# Autodesk Inventor assembly: TestAssm
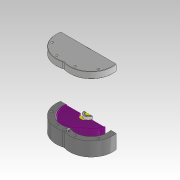
[picture p0: Inventor's stored thumbnail of the model, 180x180]
Saved by Autodesk Inventor 2020 (Build 240168000, 168)
## iProperties
Created: 2021-05-17
Part Number: TestAssm
Document SubType Name: Assembly
Designer: DDeGo
Author: DDeGo
## Documents named in this file (14)
- C:\Users\DDeGo\Documents\Drew\Projects\AirWankelEngine\cad\LiquidPiston V1\TestAssm.iam
- C:\Users\DDeGo\Documents\Drew\Projects\AirWankelEngine\cad\LiquidPiston V1\TestHousing.ipt
- C:\Users\DDeGo\Documents\Drew\Projects\AirWankelEngine\cad\LiquidPiston V1\TestRotor.ipt
- C:\Users\DDeGo\Documents\Drew\Projects\AirWankelEngine\cad\LiquidPiston V1\TestCam.ipt
- C:\Users\DDeGo\Documents\Drew\Projects\AirWankelEngine\cad\LiquidPiston V1\TestAssm\Design Accelerator\Spur Gears1.iam
- C:\Users\DDeGo\Documents\Drew\Projects\AirWankelEngine\cad\hardware\6701 bearing.ipt
- C:\Users\DDeGo\Documents\Drew\Projects\AirWankelEngine\cad\LiquidPiston V1\TestHead.ipt
- C:\Users\DDeGo\Documents\Drew\Projects\AirWankelEngine\cad\LiquidPiston V1\ApexSeal.ipt
- C:\Users\DDeGo\Documents\Drew\Projects\AirWankelEngine\cad\hardware\MR85 bearing.ipt
- C:\Users\DDeGo\Documents\Drew\Projects\AirWankelEngine\cad\LiquidPiston V1\TestRotorTeeth.ipt
- C:\Users\DDeGo\Documents\Drew\Projects\AirWankelEngine\cad\LiquidPiston V1\Flywheel.ipt
- C:\Users\DDeGo\Documents\Drew\Projects\AirWankelEngine\cad\hardware\oring_4x2x1.ipt
- C:\Users\DDeGo\Documents\Drew\Projects\AirWankelEngine\cad\hardware\2x22 pin.ipt
- C:\Users\DDeGo\Documents\Drew\Projects\AirWankelEngine\cad\LiquidPiston V1\ValveThing2.ipt
## Components (18 placed, 13 different names)
1. TestHousing:1 — Mate:2, Mate:11, Mate:14, Mate:15, Mate:20, Mate:21, Mate:65, Mate:66, Mate:67, Mate:68, Mate:69
2. TestRotor:1 — Mate:2, Mate:3, Rotation:1, Mate:5, Mate:29, Mate:30, Angle:1, Mate:42
3. TestCam:1 — Mate:3, Rotation:1, Mate:43, Mate:44, Mate:46, Mate:47, Mate:48, Flush:6
4. Spur Gears:1 [sub-assembly]
5. 6701 bearing:1 — Mate:5, Mate:42, Flush:6
6. ApexSeal:1 — Mate:11, Mate:67
7. ApexSeal:2 — Mate:14, Mate:68
8. ApexSeal:3 — Mate:15, Mate:66
9. MR85 bearing:1 — Mate:20, Mate:21, Mate:32, Mate:33
10. MR85 bearing:2 — Mate:46, Mate:48, Mate:64
11. TestRotorTeeth:1 — Mate:29, Mate:30, Angle:1
12. Flywheel:1 — Mate:32, Mate:33, Mate:45, Mate:47
13. oring_4x2x1:1 — Flush:2, Flush:3, Mate:71, Tangent:1
14. oring_4x2x1:2 — Flush:2, Mate:70, Tangent:2
15. oring_4x2x1:3 — Flush:3, Mate:72
16. 2x22 pin:1 — Mate:43, Mate:44, Mate:45
17. TestHead:1 — Mate:64, Mate:65, Mate:69, Mate:70, Mate:71, Mate:72, Tangent:1, Mate:73, Mate:74
18. ValveThing2:1 — Mate:73, Mate:74, Tangent:2
## Relationships (37: Mate 30, Flush 3, Tangent 2, RelateRotation 1, Angle 1)
- Mate:2 (-0.25 mm): TestHousing:1 ↔ TestRotor:1
- Mate:3: TestRotor:1 ↔ TestCam:1
- Rotation:1 [RelateRotation] (2 ul): TestRotor:1 ↔ TestCam:1
- Mate:5: TestRotor:1 ↔ 6701 bearing:1
- Mate:11 (0.1 mm): TestHousing:1 ↔ ApexSeal:1
- Mate:14 (0.1 mm): TestHousing:1 ↔ ApexSeal:2
- Mate:15 (0.1 mm): TestHousing:1 ↔ ApexSeal:3
- Mate:20: TestHousing:1 ↔ MR85 bearing:1
- Mate:21: TestHousing:1 ↔ MR85 bearing:1
- Mate:29: TestRotor:1 ↔ TestRotorTeeth:1
- Mate:30: TestRotor:1 ↔ TestRotorTeeth:1
- Angle:1 (0 deg): TestRotor:1 ↔ TestRotorTeeth:1
- Mate:32: MR85 bearing:1 ↔ Flywheel:1
- Mate:33: MR85 bearing:1 ↔ Flywheel:1
- Flush:2: oring_4x2x1:1 ↔ oring_4x2x1:2
- Flush:3: oring_4x2x1:1 ↔ oring_4x2x1:3
- Mate:42: TestRotor:1 ↔ 6701 bearing:1
- Mate:43: TestCam:1 ↔ 2x22 pin:1
- Mate:44: TestCam:1 ↔ 2x22 pin:1
- Mate:45: Flywheel:1 ↔ 2x22 pin:1
- Mate:46: TestCam:1 ↔ MR85 bearing:2
- Mate:47: TestCam:1 ↔ Flywheel:1
- Mate:48: TestCam:1 ↔ MR85 bearing:2
- Flush:6: TestCam:1 ↔ 6701 bearing:1
- Mate:64: MR85 bearing:2 ↔ TestHead:1
- Mate:65: TestHousing:1 ↔ TestHead:1
- Mate:66: TestHousing:1 ↔ ApexSeal:3
- Mate:67: TestHousing:1 ↔ ApexSeal:1
- Mate:68: TestHousing:1 ↔ ApexSeal:2
- Mate:69 (50 mm): TestHousing:1 ↔ TestHead:1
- Mate:70: oring_4x2x1:2 ↔ TestHead:1
- Mate:71: oring_4x2x1:1 ↔ TestHead:1
- Mate:72: oring_4x2x1:3 ↔ TestHead:1
- Tangent:1: oring_4x2x1:1 ↔ TestHead:1
- Mate:73: TestHead:1 ↔ ValveThing2:1
- Mate:74: TestHead:1 ↔ ValveThing2:1
- Tangent:2: oring_4x2x1:2 ↔ ValveThing2:1
